# Autodesk Inventor assembly: Platevergleich
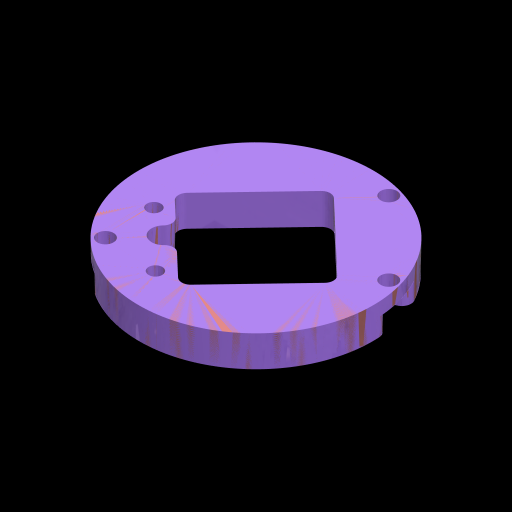
[picture p0: Inventor's stored thumbnail of the model, 512x512]
Saved by Autodesk Inventor 2024 (Build 280153000, 153)
## iProperties
Created: 2023-06-26
Part Number: Platevergleich
Document SubType Name: Assembly
Designer: buchmannmartin
Author: buchmannmartin
## Documents named in this file (3)
- E:\User\Dokumente\#BeneEspressoscope\Platevergleich.iam
- E:\User\Dokumente\#BeneEspressoscope\Assembly_Matchboxscope_injectionmolded_IM_Matchboxscope_plate_2.ipt
- E:\User\Dokumente\#BeneEspressoscope\Assembly_Matchboxscope_injectionmolded_IM_Matchboxscope_plate_3.ipt
## Components (2 placed, 2 different names)
1. Assembly_Matchboxscope_injectionmolded_IM_Matchboxscope_plate_2:1 — Fluchtend:1, Passend:1, Winkel:1
2. Assembly_Matchboxscope_injectionmolded_IM_Matchboxscope_plate_3:1 — Fluchtend:1, Passend:1, Winkel:1
## Relationships (3: Flush 1, Mate 1, Angle 1)
- Fluchtend:1 [Flush]: Assembly_Matchboxscope_injectionmolded_IM_Matchboxscope_plate_2:1 ↔ Assembly_Matchboxscope_injectionmolded_IM_Matchboxscope_plate_3:1
- Passend:1 [Mate]: Assembly_Matchboxscope_injectionmolded_IM_Matchboxscope_plate_2:1 ↔ Assembly_Matchboxscope_injectionmolded_IM_Matchboxscope_plate_3:1
- Winkel:1 [Angle] (0 deg): Assembly_Matchboxscope_injectionmolded_IM_Matchboxscope_plate_2:1 ↔ Assembly_Matchboxscope_injectionmolded_IM_Matchboxscope_plate_3:1
